# Autodesk Inventor assembly: EnsamblajeMoto
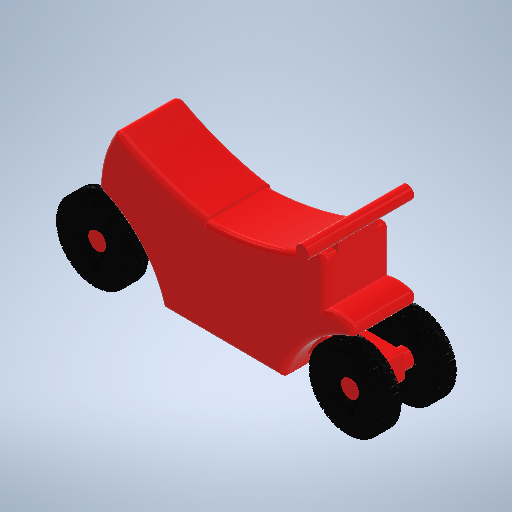
[picture p0: Inventor's stored thumbnail of the model, 512x512]
Saved by Autodesk Inventor 2025.1 (Build 291241000, 241)
## iProperties
Created: 2025-01-19
Part Number: EnsamblajeMoto
Document SubType Name: Assembly
Designer: usuario
Author: usuario
## Documents named in this file (4)
- C:\Users\yovan\Desktop\APM\ausol-apm.github.io\project\Design and simulation\Inventor\Modelado juguetes\Moto\EnsamblajeMotoFinal.iam
- C:\Users\yovan\Desktop\APM\ausol-apm.github.io\project\Design and simulation\Inventor\Modelado juguetes\Moto\PiezaParteAtrasMoto.ipt
- C:\Users\yovan\Desktop\APM\ausol-apm.github.io\project\Design and simulation\Inventor\Modelado juguetes\Moto\PiezaParteDelanteraMoto.ipt
- C:\Users\yovan\Desktop\APM\ausol-apm.github.io\project\Design and simulation\Inventor\Modelado juguetes\Moto\Llanta.ipt
## Components (6 placed, 3 different names)
1. PiezaParteAtrasMoto:1 — Mate:1, Flush:1, Flush:2, Mate:2, Mate:4, Flush:3, Flush:6
2. PiezaParteDelanteraMoto:1 — Mate:1, Flush:1, Flush:2, Mate:3, Mate:5, Flush:4, Flush:5
3. Llanta:1 — Mate:2, Flush:3
4. Llanta:2 — Mate:4, Flush:6
5. Llanta:3 — Mate:3, Flush:4
6. Llanta:4 — Mate:5, Flush:5
## Relationships (11: Flush 6, Mate 5)
- Mate:1: PiezaParteAtrasMoto:1 ↔ PiezaParteDelanteraMoto:1
- Flush:1: PiezaParteAtrasMoto:1 ↔ PiezaParteDelanteraMoto:1
- Flush:2: PiezaParteAtrasMoto:1 ↔ PiezaParteDelanteraMoto:1
- Mate:2: PiezaParteAtrasMoto:1 ↔ Llanta:1
- Mate:3: PiezaParteDelanteraMoto:1 ↔ Llanta:3
- Mate:4: PiezaParteAtrasMoto:1 ↔ Llanta:2
- Mate:5: PiezaParteDelanteraMoto:1 ↔ Llanta:4
- Flush:3: PiezaParteAtrasMoto:1 ↔ Llanta:1
- Flush:4: PiezaParteDelanteraMoto:1 ↔ Llanta:3
- Flush:5: PiezaParteDelanteraMoto:1 ↔ Llanta:4
- Flush:6: PiezaParteAtrasMoto:1 ↔ Llanta:2
